# Autodesk Inventor assembly: right pneumatics board
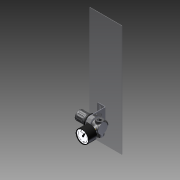
[picture p0: Inventor's stored thumbnail of the model, 180x180]
Saved by Autodesk Inventor 2014 SP1 (Build 180222100, 222)
## iProperties
Created: 2014-01-20
Part Number: right pneumatics board
Document SubType Name: Assembly
Designer: Arpan
Author: Arpan
## Documents named in this file (3)
- C:\Users\Arpan\Documents\GitHub\2014buildCAD\pneumatics board\right pneumatics board.iam
- C:\Users\Arpan\Documents\GitHub\2014buildCAD\pneumatics board\pneumatics board 1.ipt
- C:\Users\Arpan\Documents\GitHub\2014buildCAD\pneumatics board\pneumatics thing 2.iam
## Components (2 placed, 2 different names)
1. pneumatics board 1:1 — Mate:1
2. pneumatics thing 2:1 [sub-assembly] — Mate:1
## Relationships (1: Mate 1)
- Mate:1: pneumatics board 1:1 ↔ pneumatics thing 2:1
